# Autodesk Inventor assembly: Final Leg Assembly
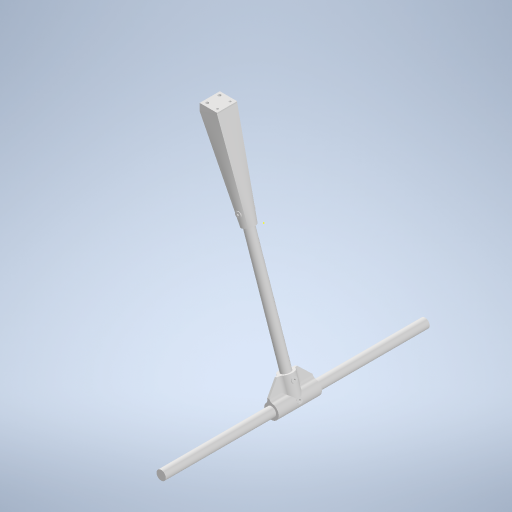
[picture p0: Inventor's stored thumbnail of the model, 512x512]
Saved by Autodesk Inventor 2023 (Build 270158000, 158)
## iProperties
Created: 2023-01-18
Part Number: Final Leg Assembly
Document SubType Name: Assembly
Designer: chase
Author: chase
## Documents named in this file (5)
- C:\Users\chase\Desktop\Senior Project\Final Leg Assembly.iam
- C:\Users\chase\OneDrive\Documents\GitHub\WU-Team20-AutonomousDrone\CAD\Legs\UpperLandingLegMount3.ipt
- C:\Users\chase\Downloads\16mm leg.ipt
- C:\Users\chase\OneDrive\Documents\GitHub\WU-Team20-AutonomousDrone\CAD\Legs\LegTeeJoint2.5.ipt
- C:\Users\chase\OneDrive\Documents\GitHub\WU-Team20-AutonomousDrone\CAD\Legs\Landing Foot.ipt
## Components (4 placed, 4 different names)
1. UpperLandingLegMount3:1 — Insert:1
2. 16mm leg:1 — Insert:1, Insert:2
3. LegTeeJoint2.5:1 — Insert:2, Insert:3
4. Landing Foot:1 — Insert:3
## Relationships (3: Insert 3)
- Insert:1: UpperLandingLegMount3:1 ↔ 16mm leg:1
- Insert:2: 16mm leg:1 ↔ LegTeeJoint2.5:1
- Insert:3 (-191.1 mm): LegTeeJoint2.5:1 ↔ Landing Foot:1
